# Autodesk Inventor assembly: ChessBoard
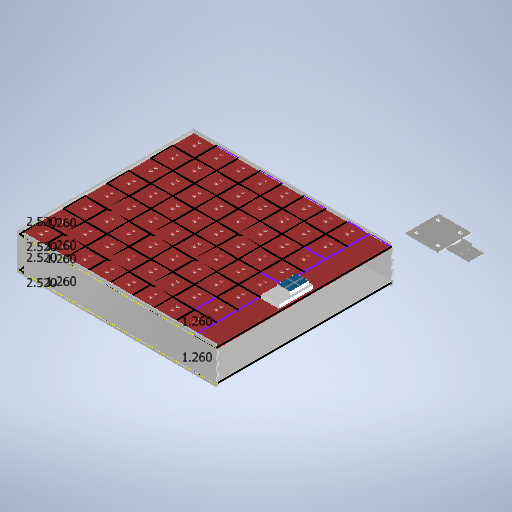
[picture p0: Inventor's stored thumbnail of the model, 512x512]
Saved by Autodesk Inventor 2025.2 (Build 292293000, 293)
## iProperties
Created: 2025-04-21
Part Number: ChessBoard
Document SubType Name: Assembly
Designer: powel
Author: powel
## Documents named in this file (9)
- C:\Users\powel\Desktop\School\24-25\Spring\Chess Set\ChessBoard.iam
- C:\Users\powel\Desktop\School\24-25\Spring\Chess Set\LED Holder.ipt
- C:\Users\powel\Desktop\School\24-25\Spring\Chess Set\Side Wall.ipt
- C:\Users\powel\Desktop\School\24-25\Spring\Chess Set\Floor.ipt
- C:\Users\powel\Desktop\School\24-25\Spring\Chess Set\Side Wall 3.ipt
- C:\Users\powel\Desktop\School\24-25\Spring\Chess Set\Side Wall_MIR1.ipt
- C:\Users\powel\Desktop\School\24-25\Spring\Chess Set\Wire Position.ipt
- C:\Users\powel\Desktop\School\24-25\Spring\Chess Set\LED Position.ipt
- C:\Users\powel\Desktop\School\24-25\Spring\Chess Set\Wall Test.ipt
## Components (9 placed, 8 different names)
1. LED Holder:1 — Rigid:10
2. Side Wall:1 — Rigid:9, Rigid:10, Rigid:12
3. Floor:1 — Rigid:9, Rigid:11
4. Floor:2 — Rigid:13
5. Side Wall 3:1 — Rigid:12
6. Side Wall 2:1 — Rigid:11, Rigid:13
7. Wire Position:1
8. LED Position:1
9. Wall Test:1
## Relationships (5: WeldJoint 5)
- Rigid:9 [WeldJoint]: Side Wall:1 ↔ Floor:1
- Rigid:10 [WeldJoint]: LED Holder:1 ↔ Side Wall:1
- Rigid:11 [WeldJoint]: Floor:1 ↔ Side Wall 2:1
- Rigid:12 [WeldJoint]: Side Wall:1 ↔ Side Wall 3:1
- Rigid:13 [WeldJoint]: Floor:2 ↔ Side Wall 2:1
## Named parameters: Finish10_Area = 349.292, Finish11_Area = 2140.26, Finish1_Area = 3355.99, Finish2_Area = 5.06317, Finish3_Area = 20.1946, Finish4_Area = 1502.2, Finish5_Area = 638.065, Finish6_Area = 1509.57, Finish7_Area = 5.06317, Finish8_Area = 20.1946, Finish9_Area = 1502.2
note: some values were not read from the file. Shown as the stored number, unit unknown: "Finish10_Area", "Finish11_Area", "Finish1_Area", "Finish2_Area", "Finish3_Area", "Finish4_Area", "Finish5_Area", "Finish6_Area", "Finish7_Area", "Finish8_Area", "Finish9_Area".
